# Autodesk Inventor assembly: shaft assembly
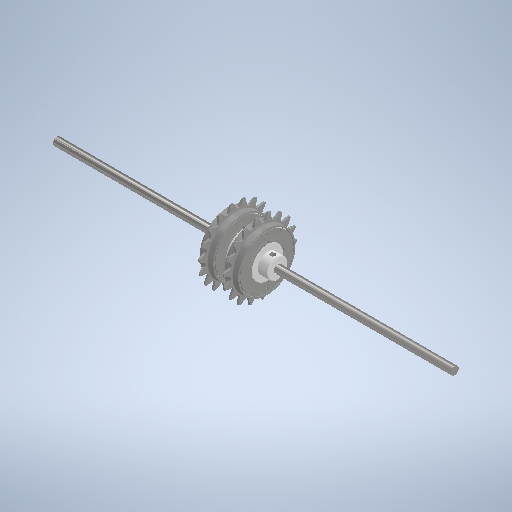
[picture p0: Inventor's stored thumbnail of the model, 512x512]
Saved by Autodesk Inventor 2026.1 (Build 301233020, 233B)
## iProperties
Created: 2026-01-22
Part Number: shaft assembly
Document SubType Name: Assembly
Designer: user
Author: user
## Documents named in this file (4)
- D:\asu\machine element design\project\design\shaft assembly.iam
- C:\Users\user\Downloads\18t_single-speed_freewheel-1.snapshot.1\18T_ss_fw\18T_ss_fw\18T_ss_fw.iam
- D:\asu\machine element design\project\design\shaft.ipt
- D:\asu\machine element design\project\design\sprocet adaptor2.ipt
## Components (4 placed, 3 different names)
1. shaft:1 — Mate:5
2. 18T_ss_fw:1 [sub-assembly] — Mate:1, Mate:2
3. 18T_ss_fw:2 [sub-assembly] — Mate:3, Mate:4
4. sprocet adaptor2:1 — Mate:1, Mate:2, Mate:3, Mate:4, Mate:5
## Relationships (5: Mate 5)
- Mate:1: 18T_ss_fw:1 ↔ sprocet adaptor2:1
- Mate:2: 18T_ss_fw:1 ↔ sprocet adaptor2:1
- Mate:3: 18T_ss_fw:2 ↔ sprocet adaptor2:1
- Mate:4: 18T_ss_fw:2 ↔ sprocet adaptor2:1
- Mate:5: shaft:1 ↔ sprocet adaptor2:1
